# Autodesk Inventor assembly: PIHTI-for-Boron_Hayashi
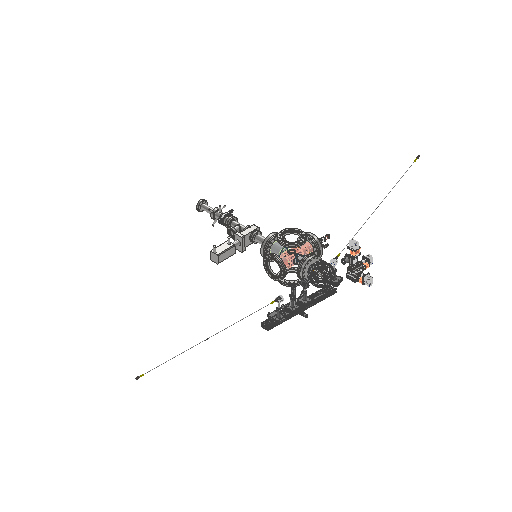
[picture p0: Inventor's stored thumbnail of the model, 512x512]
Saved by Autodesk Inventor 2026.2 (Build 302298000, 298)
## iProperties
Created: 2024-05-09
Part Number: PIHTI-for-Boron_Hayashi
Document SubType Name: Assembly
Designer: kuzmin
Mass: 19614.5 g
Surface Area: 13609.5 cm^2
Volume: 3689.47 cm^3
Density: 5.31636 g/cm^3
Author: kuzmin
## Documents named in this file (25)
- D:\repos\PIHTI\Plasma Vessel_2026\PIHTI-for-Boron_Hayashi.iam
- D:\repos\PIHTI\Plasma Vessel\Plasma-vacuum-cross\Plasma-vacuum-vessel-152IC-cross.iam
- D:\repos\PIHTI\Plasma Vessel\Plasma-Box\Plasma-box-hayashi-aka-upgrade.iam
- D:\repos\PIHTI\ContentCenter\Fastners\M3x8-SHCS.ipt
- D:\repos\PIHTI\Plasma Vessel\Plasma-Box\probe-gate-with-spindel.iam
- D:\repos\PIHTI\Plasma Vessel\Cathode-Anode-Flange\cf70_spacer.ipt
- D:\repos\PIHTI\Plasma Vessel\entrance-mesh-assembly.iam
- D:\repos\PIHTI\Plasma Vessel\probe-port-mesh-welded.iam
- D:\repos\PIHTI\ContentCenter\CF-parts\CF70-nipple\CF70-nipple.iam
- D:\repos\PIHTI\ContentCenter\CF-parts\CF70-gate-valve\Gatevalve_70_pneumatic.iam
- D:\repos\PIHTI\Plasma Vessel_2026\contents\CF-70-Tee.ipt
- D:\repos\PIHTI\Plasma Vessel_2026\contents\ICF70_to_KF40.ipt
- D:\repos\PIHTI\Plasma Vessel_2026\Cathode-Anode-Flange\Cathode-Anode-70IC-flange-with-feeds.iam
- D:\repos\PIHTI\Plasma Vessel_2026\Plasma-Flange-2024\cathode-box-on-a-flange.iam
- D:\repos\PIHTI\Plasma Vessel_2026\contents\NW40_viton_centering_ring.ipt
- D:\repos\PIHTI\Plasma Vessel_2026\contents\NW40_clamp.ipt
- D:\repos\PIHTI\Plasma Vessel_2026\contents\CF_152-70_bearing.ipt
- D:\repos\PIHTI\Plasma Vessel_2026\contents\B_probe_bearing.ipt
- D:\repos\PIHTI\Plasma Vessel_2026\contents\M4×12-VentedHexBolt.ipt
- D:\repos\PIHTI\Plasma Vessel_2026\contents\OringFixture.iam
- D:\repos\PIHTI\Plasma Vessel_2026\Plasma-vacuum-vessel\Plasma-vacuum-vessel-34IC-cross.iam
- D:\repos\PIHTI\SpectroscopySystem_Hayashi\ラマン分光系.iam
- D:\repos\PIHTI\SpectroscopySystem_Hayashi\LIBS分光系.iam
- D:\repos\PIHTI\SpectroscopySystem_Hayashi\Optics\LIBSコリメータ.iam
- D:\repos\PIHTI\BoronProbe\palp-boron-hybrid.iam
## Components (34 placed, 24 different names)
1. Plasma-vacuum-vessel-152IC-cross:1 [sub-assembly] — メイト:1, フラッシュ:1, フラッシュ:2, リジッド:18, メイト:59, メイト:60, メイト:83, メイト:84, メイト:85, 角度:2, メイト:90
2. Plasma-box-hayashi-aka-upgrade:1 [sub-assembly] — メイト:3, メイト:4, Hinge Angle, メイト:13, メイト:17
3. probe-gate-with-spindel:1 [sub-assembly] — メイト:3, メイト:4, Hinge Angle
4. cf70_spacer:1 — メイト:61, メイト:62, メイト:63, メイト:64
5. entrance-mesh-assembly:1 [sub-assembly] — メイト:13, メイト:17, メイト:19
6. probe-port-mesh-welded:1 [sub-assembly] — メイト:19
7. CF_152-70_bearing:1 — リジッド:18, リジッド:21, メイト:72, メイト:73, メイト:74
8. CF70-nipple:1 [sub-assembly] — リジッド:21, リジッド:22
9. Gatevalve_70_pneumatic:1 [sub-assembly] — リジッド:22, メイト:47, メイト:48, メイト:49
10. CF-70-Tee:1 — メイト:47, メイト:48, メイト:49, メイト:50, メイト:51, メイト:52
11. ICF70_to_KF40:1 — メイト:50, メイト:51, メイト:52, メイト:67, メイト:68, メイト:70, メイト:71
12. Cathode-Anode-70IC-flange-with-feeds:1 [sub-assembly] — メイト:63, メイト:64
13. cathode-box-on-a-flange:1 [sub-assembly] — メイト:59, メイト:60, メイト:61, メイト:62
14. NW40_viton_centering_ring:1 — メイト:67, メイト:68, メイト:81, メイト:82
15. NW40_clamp:1 — メイト:70, メイト:71
16. B_probe_bearing:1 — メイト:72, メイト:73, メイト:74, メイト:75, メイト:76, メイト:77, メイト:78, メイト:79, メイト:80
17. M4×12-VentedHexBolt:1 — メイト:75, メイト:76
18. M4×12-VentedHexBolt:2 — メイト:77, メイト:78
19. M4×12-VentedHexBolt:3 — メイト:79, メイト:80
20. OringFixture:1 [sub-assembly] — メイト:81, メイト:82, メイト:91
21. CF_152-70_bearing:2 — メイト:83, メイト:84, メイト:85, メイト:86, メイト:87
22. Plasma-vacuum-vessel-34IC-cross:1 [sub-assembly] — メイト:86, メイト:87, 角度:2, メイト:88, 角度:3, メイト:89, 角度:4
23. ラマン分光系:1 [sub-assembly] — メイト:88, 角度:3
24. LIBS分光系:1 [sub-assembly] — メイト:89, 角度:4, 角度:5, フラッシュ:7
25. palp-boron-hybrid:1 [sub-assembly] — メイト:90, メイト:91
26. LIBSコリメータ:1 [sub-assembly] — 角度:5, フラッシュ:7
27. SS ISO 4762 M3 x 8:5
28. SS ISO 4762 M3 x 8:6
29. SS ISO 4762 M3 x 8:7
30. SS ISO 4762 M3 x 8:8
31. SS ISO 4762 M3 x 8:1
32. SS ISO 4762 M3 x 8:2
33. SS ISO 4762 M3 x 8:3
34. SS ISO 4762 M3 x 8:4
## Relationships (53: Mate 42, Angle 5, Flush 3, WeldJoint 3)
- メイト:1 [Mate]: Plasma-vacuum-vessel-152IC-cross:1
- フラッシュ:1 [Flush]: Plasma-vacuum-vessel-152IC-cross:1
- フラッシュ:2 [Flush]: Plasma-vacuum-vessel-152IC-cross:1
- メイト:3 [Mate]: Plasma-box-hayashi-aka-upgrade:1 ↔ probe-gate-with-spindel:1
- メイト:4 [Mate]: Plasma-box-hayashi-aka-upgrade:1 ↔ probe-gate-with-spindel:1
- Hinge Angle [Angle] (45 deg): Plasma-box-hayashi-aka-upgrade:1 ↔ probe-gate-with-spindel:1
- メイト:13 [Mate]: Plasma-box-hayashi-aka-upgrade:1 ↔ entrance-mesh-assembly:1
- メイト:17 [Mate]: Plasma-box-hayashi-aka-upgrade:1 ↔ entrance-mesh-assembly:1
- メイト:19 [Mate]: entrance-mesh-assembly:1 ↔ probe-port-mesh-welded:1
- リジッド:18 [WeldJoint]: Plasma-vacuum-vessel-152IC-cross:1 ↔ CF_152-70_bearing:1
- リジッド:21 [WeldJoint]: CF_152-70_bearing:1 ↔ CF70-nipple:1
- リジッド:22 [WeldJoint]: CF70-nipple:1 ↔ Gatevalve_70_pneumatic:1
- メイト:47 [Mate]: Gatevalve_70_pneumatic:1 ↔ CF-70-Tee:1
- メイト:48 [Mate]: Gatevalve_70_pneumatic:1 ↔ CF-70-Tee:1
- メイト:49 [Mate]: Gatevalve_70_pneumatic:1 ↔ CF-70-Tee:1
- メイト:50 [Mate]: CF-70-Tee:1 ↔ ICF70_to_KF40:1
- メイト:51 [Mate]: CF-70-Tee:1 ↔ ICF70_to_KF40:1
- メイト:52 [Mate]: CF-70-Tee:1 ↔ ICF70_to_KF40:1
- メイト:59 [Mate]: Plasma-vacuum-vessel-152IC-cross:1 ↔ cathode-box-on-a-flange:1
- メイト:60 [Mate]: Plasma-vacuum-vessel-152IC-cross:1 ↔ cathode-box-on-a-flange:1
- メイト:61 [Mate]: cf70_spacer:1 ↔ cathode-box-on-a-flange:1
- メイト:62 [Mate]: cf70_spacer:1 ↔ cathode-box-on-a-flange:1
- メイト:63 [Mate]: cf70_spacer:1 ↔ Cathode-Anode-70IC-flange-with-feeds:1
- メイト:64 [Mate]: cf70_spacer:1 ↔ Cathode-Anode-70IC-flange-with-feeds:1
- メイト:67 [Mate]: ICF70_to_KF40:1 ↔ NW40_viton_centering_ring:1
- メイト:68 [Mate]: ICF70_to_KF40:1 ↔ NW40_viton_centering_ring:1
- メイト:70 [Mate]: ICF70_to_KF40:1 ↔ NW40_clamp:1
- メイト:71 [Mate]: ICF70_to_KF40:1 ↔ NW40_clamp:1
- メイト:72 [Mate]: CF_152-70_bearing:1 ↔ B_probe_bearing:1
- メイト:73 [Mate]: CF_152-70_bearing:1 ↔ B_probe_bearing:1
- メイト:74 [Mate]: CF_152-70_bearing:1 ↔ B_probe_bearing:1
- メイト:75 [Mate]: B_probe_bearing:1 ↔ M4×12-VentedHexBolt:1
- メイト:76 [Mate]: B_probe_bearing:1 ↔ M4×12-VentedHexBolt:1
- メイト:77 [Mate]: B_probe_bearing:1 ↔ M4×12-VentedHexBolt:2
- メイト:78 [Mate]: B_probe_bearing:1 ↔ M4×12-VentedHexBolt:2
- メイト:79 [Mate]: B_probe_bearing:1 ↔ M4×12-VentedHexBolt:3
- メイト:80 [Mate]: B_probe_bearing:1 ↔ M4×12-VentedHexBolt:3
- メイト:81 [Mate]: NW40_viton_centering_ring:1 ↔ OringFixture:1
- メイト:82 [Mate]: NW40_viton_centering_ring:1 ↔ OringFixture:1
- メイト:83 [Mate]: Plasma-vacuum-vessel-152IC-cross:1 ↔ CF_152-70_bearing:2
- メイト:84 [Mate]: Plasma-vacuum-vessel-152IC-cross:1 ↔ CF_152-70_bearing:2
- メイト:85 [Mate]: Plasma-vacuum-vessel-152IC-cross:1 ↔ CF_152-70_bearing:2
- メイト:86 [Mate]: CF_152-70_bearing:2 ↔ Plasma-vacuum-vessel-34IC-cross:1
- メイト:87 [Mate]: CF_152-70_bearing:2 ↔ Plasma-vacuum-vessel-34IC-cross:1
- 角度:2 [Angle] (0 deg): Plasma-vacuum-vessel-152IC-cross:1 ↔ Plasma-vacuum-vessel-34IC-cross:1
- メイト:88 [Mate]: Plasma-vacuum-vessel-34IC-cross:1 ↔ ラマン分光系:1
- 角度:3 [Angle] (0 deg): Plasma-vacuum-vessel-34IC-cross:1 ↔ ラマン分光系:1
- メイト:89 [Mate]: Plasma-vacuum-vessel-34IC-cross:1 ↔ LIBS分光系:1
- 角度:4 [Angle] (0 deg): Plasma-vacuum-vessel-34IC-cross:1 ↔ LIBS分光系:1
- メイト:90 [Mate]: Plasma-vacuum-vessel-152IC-cross:1 ↔ palp-boron-hybrid:1
- メイト:91 [Mate] (90 mm): OringFixture:1 ↔ palp-boron-hybrid:1
- 角度:5 [Angle] (20 deg): LIBS分光系:1 ↔ LIBSコリメータ:1
- フラッシュ:7 [Flush] (-25 mm): LIBS分光系:1 ↔ LIBSコリメータ:1
## Named parameters: ProbePos = 90 mm, ProbePos_Max = 90 mm, ProbePos_Min = 308 mm, ProbePos_Ext = 920 mm
